# Autodesk Inventor assembly: Сборка апрель
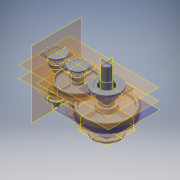
[picture p0: Inventor's stored thumbnail of the model, 180x180]
Saved by Autodesk Inventor 2018 (Build 220112000, 112)
## iProperties
Created: 2018-03-25
Part Number: Сборка апрель
Material: Типовые
Document SubType Name: Assembly
Designer: kriku
Mass: 4694.56 g
Surface Area: 6620.58 cm^2
Volume: 2953.87 cm^3
Density: 1.58929 g/cm^3
Author: kriku
## Documents named in this file (21)
- C:\Users\kriku\OneDrive\Рабочий стол\6 семестр\курсач ДМ\deadmash\Куча инви\Сборка апрель.iam
- C:\Users\kriku\OneDrive\Рабочий стол\6 семестр\курсач ДМ\deadmash\Куча инви\Вал быстроходный.ipt
- C:\Users\kriku\OneDrive\Рабочий стол\6 семестр\курсач ДМ\deadmash\Куча инви\Колесо быстроходное.ipt
- C:\Users\kriku\OneDrive\Рабочий стол\6 семестр\курсач ДМ\deadmash\Куча инви\Вал переходный.ipt
- C:\Users\kriku\OneDrive\Рабочий стол\6 семестр\курсач ДМ\deadmash\Куча инви\Колесл тихоходное.ipt
- C:\Users\kriku\OneDrive\Рабочий стол\6 семестр\курсач ДМ\deadmash\Куча инви\Вал тихоходный.ipt
- C:\Users\kriku\OneDrive\Документы\Inventor\Content Center Files\R2018\ru-RU\GOST 8338-75\Подшипник 206 ГОСТ 8338-75.ipt
- C:\Users\kriku\OneDrive\Документы\Inventor\Content Center Files\R2018\ru-RU\GOST 8338-75\Подшипник 211 ГОСТ 8338-75.ipt
- C:\Users\kriku\OneDrive\Рабочий стол\6 семестр\курсач ДМ\deadmash\Куча инви\Сборка1\Мастер проектирования\Шпоночное соединение1.iam
- C:\Users\kriku\OneDrive\Рабочий стол\6 семестр\курсач ДМ\Куча инви\Крышка обычная на 30.ipt
- C:\Users\kriku\OneDrive\Рабочий стол\6 семестр\курсач ДМ\Куча инви\Крышка обычная на 55.ipt
- C:\Users\kriku\OneDrive\Рабочий стол\6 семестр\курсач ДМ\Куча инви\Крышка сквозная на 55.ipt
- C:\Users\kriku\OneDrive\Документы\Inventor\Content Center Files\R2018\ru-RU\GOST 8752-79(1)\Манжет 1-55x80x8 ГОСТ 8752-79.ipt
- C:\Users\kriku\OneDrive\Рабочий стол\6 семестр\курсач ДМ\Куча инви\Крышка сквозная на 30.ipt
- C:\Users\kriku\OneDrive\Документы\Inventor\Content Center Files\R2018\ru-RU\GOST 8752-79(1)\Манжет 1-30x47x7 ГОСТ 8752-79.ipt
- C:\Users\kriku\OneDrive\Рабочий стол\6 семестр\курсач ДМ\Куча инви\заплечик быстроход больший.ipt
- C:\Users\kriku\OneDrive\Рабочий стол\6 семестр\курсач ДМ\Куча инви\заплечик быстроход меньший.ipt
- C:\Users\kriku\OneDrive\Рабочий стол\6 семестр\курсач ДМ\Куча инви\заплечик переходный.ipt
- C:\Users\kriku\OneDrive\Рабочий стол\6 семестр\курсач ДМ\Куча инви\заплечик переходный  кряком.ipt
- C:\Users\kriku\OneDrive\Рабочий стол\6 семестр\курсач ДМ\Куча инви\заплечикбыстроходный  кряком.ipt
- C:\Users\kriku\OneDrive\Рабочий стол\6 семестр\курсач ДМ\Куча инви\плюс к быстроходному.ipt
## Components (26 placed, 20 different names)
1. Вал быстроходный:1 — Совмещение:1, Совмещение:2, Совмещение:11, Совмещение:12, Совмещение:17, Совмещение:20, Заподлицо:7, Заподлицо:8, Заподлицо:10, Совмещение:36, Цилиндрический:1, Жесткий:1
2. Колесо быстроходное:1 — Заподлицо:1, Совмещение:1, Совмещение:2, Совмещение:3, Совмещение:4, Совмещение:5, Угол:2, С поворотом:5
3. Вал переходный:1 — Совмещение:3, Совмещение:4, Совмещение:5, Совмещение:6, Совмещение:7, Совмещение:8, Совмещение:13, Совмещение:14, Совмещение:18, Совмещение:23, Заподлицо:3, Угол:1, Совмещение:24, Угол:2, Заподлицо:4, Заподлицо:5, Совмещение:26, Заподлицо:6, Совмещение:32, Совмещение:33, Вставка:1
4. Колесл тихоходное:1 — Совмещение:6, Совмещение:7, Совмещение:8, Совмещение:9, Заподлицо:2, Совмещение:10, Совмещение:32, Совмещение:33, С поворотом:3
5. Вал тихоходный:1 — Совмещение:9, Заподлицо:2, Совмещение:10, Совмещение:15, Совмещение:16, Совмещение:19, Совмещение:22, Совмещение:29, Совмещение:30, Совмещение:34, Заподлицо:9
6. Подшипник ГОСТ 8338-75 206:1 — Совмещение:11, Совмещение:17, Совмещение:28, Совмещение:38
7. Подшипник ГОСТ 8338-75 206:2 — Совмещение:12, Совмещение:20, Совмещение:37
8. Подшипник ГОСТ 8338-75 206:3 — Совмещение:13, Совмещение:18, Совмещение:25
9. Подшипник ГОСТ 8338-75 206:4 — Совмещение:14, Совмещение:23, Совмещение:27
10. Подшипник ГОСТ 8338-75 211:1 — Совмещение:15, Совмещение:22, Совмещение:31, С поворотом:4
11. Подшипник ГОСТ 8338-75 211:2 — Совмещение:16, Совмещение:19, Совмещение:35
12. Шпоночное соединение:1 [sub-assembly] — Заподлицо:3, Угол:1, Совмещение:24
13. Крышка обычная на 30:1 — Заподлицо:4, Заподлицо:5, Совмещение:25
14. Крышка обычная на 30:2 — Совмещение:26, Заподлицо:6, Совмещение:27
15. Крышка обычная на 30:3 — Заподлицо:7, Заподлицо:8, Совмещение:28
16. Крышка обычная на 55:1 — Совмещение:29, Совмещение:30, Совмещение:31
17. Крышка сквозная на 55:1 — Совмещение:34, Заподлицо:9, С поворотом:1, Совмещение:35
18. Манжет 1 ГОСТ 8752-79 55 x 80 x 8:1 — С поворотом:1
19. Крышка сквозная на 30:1 — С поворотом:2, Заподлицо:10, Совмещение:36, Совмещение:37
20. Манжет 1 ГОСТ 8752-79 30 x 47 x 7:1 — С поворотом:2
21. заплечик быстроход больший:1 — С поворотом:3
22. заплечик быстроход меньший:1 — С поворотом:4
23. заплечик переходный:1 — С поворотом:5
24. заплечик переходный  кряком:1 — Вставка:1
25. заплечикбыстроходный  кряком:1 — Совмещение:38, Цилиндрический:1
26. плюс к быстроходному:1 — Жесткий:1
## Relationships (58: Mate 37, Flush 11, RevoluteJoint 5, Angle 2, Insert 1, CylindricalJoint 1, WeldJoint 1)
- Заподлицо:1 [Flush]: Колесо быстроходное:1
- Совмещение:1 [Mate] (110 mm): Вал быстроходный:1 ↔ Колесо быстроходное:1
- Совмещение:2 [Mate]: Вал быстроходный:1 ↔ Колесо быстроходное:1
- Совмещение:3 [Mate]: Колесо быстроходное:1 ↔ Вал переходный:1
- Совмещение:4 [Mate]: Колесо быстроходное:1 ↔ Вал переходный:1
- Совмещение:5 [Mate]: Колесо быстроходное:1 ↔ Вал переходный:1
- Совмещение:6 [Mate]: Вал переходный:1 ↔ Колесл тихоходное:1
- Совмещение:7 [Mate]: Вал переходный:1 ↔ Колесл тихоходное:1
- Совмещение:8 [Mate] (150 mm): Вал переходный:1 ↔ Колесл тихоходное:1
- Совмещение:9 [Mate]: Колесл тихоходное:1 ↔ Вал тихоходный:1
- Заподлицо:2 [Flush]: Колесл тихоходное:1 ↔ Вал тихоходный:1
- Совмещение:10 [Mate] (11 mm): Колесл тихоходное:1 ↔ Вал тихоходный:1
- Совмещение:11 [Mate]: Вал быстроходный:1 ↔ Подшипник ГОСТ 8338-75 206:1
- Совмещение:12 [Mate]: Вал быстроходный:1 ↔ Подшипник ГОСТ 8338-75 206:2
- Совмещение:13 [Mate]: Вал переходный:1 ↔ Подшипник ГОСТ 8338-75 206:3
- Совмещение:14 [Mate]: Вал переходный:1 ↔ Подшипник ГОСТ 8338-75 206:4
- Совмещение:15 [Mate]: Вал тихоходный:1 ↔ Подшипник ГОСТ 8338-75 211:1
- Совмещение:16 [Mate]: Вал тихоходный:1 ↔ Подшипник ГОСТ 8338-75 211:2
- Совмещение:17 [Mate]: Вал быстроходный:1 ↔ Подшипник ГОСТ 8338-75 206:1
- Совмещение:18 [Mate]: Вал переходный:1 ↔ Подшипник ГОСТ 8338-75 206:3
- Совмещение:19 [Mate]: Вал тихоходный:1 ↔ Подшипник ГОСТ 8338-75 211:2
- Совмещение:20 [Mate]: Вал быстроходный:1 ↔ Подшипник ГОСТ 8338-75 206:2
- Совмещение:22 [Mate]: Вал тихоходный:1 ↔ Подшипник ГОСТ 8338-75 211:1
- Совмещение:23 [Mate]: Вал переходный:1 ↔ Подшипник ГОСТ 8338-75 206:4
- Заподлицо:3 [Flush] (16 mm): Вал переходный:1 ↔ Шпоночное соединение:1
- Угол:1 [Angle] (180 deg): Вал переходный:1 ↔ Шпоночное соединение:1
- Совмещение:24 [Mate]: Вал переходный:1 ↔ Шпоночное соединение:1
- Угол:2 [Angle] (90 deg): Колесо быстроходное:1 ↔ Вал переходный:1
- Заподлицо:4 [Flush]: Вал переходный:1 ↔ Крышка обычная на 30:1
- Заподлицо:5 [Flush]: Вал переходный:1 ↔ Крышка обычная на 30:1
- Совмещение:25 [Mate]: Подшипник ГОСТ 8338-75 206:3 ↔ Крышка обычная на 30:1
- Совмещение:26 [Mate]: Вал переходный:1 ↔ Крышка обычная на 30:2
- Заподлицо:6 [Flush]: Вал переходный:1 ↔ Крышка обычная на 30:2
- Совмещение:27 [Mate]: Подшипник ГОСТ 8338-75 206:4 ↔ Крышка обычная на 30:2
- Заподлицо:7 [Flush]: Вал быстроходный:1 ↔ Крышка обычная на 30:3
- Заподлицо:8 [Flush]: Вал быстроходный:1 ↔ Крышка обычная на 30:3
- Совмещение:28 [Mate]: Подшипник ГОСТ 8338-75 206:1 ↔ Крышка обычная на 30:3
- Совмещение:29 [Mate]: Вал тихоходный:1 ↔ Крышка обычная на 55:1
- Совмещение:30 [Mate]: Вал тихоходный:1 ↔ Крышка обычная на 55:1
- Совмещение:31 [Mate]: Подшипник ГОСТ 8338-75 211:1 ↔ Крышка обычная на 55:1
- Совмещение:32 [Mate]: Вал переходный:1 ↔ Колесл тихоходное:1
- Совмещение:33 [Mate]: Вал переходный:1 ↔ Колесл тихоходное:1
- Совмещение:34 [Mate]: Вал тихоходный:1 ↔ Крышка сквозная на 55:1
- Заподлицо:9 [Flush]: Вал тихоходный:1 ↔ Крышка сквозная на 55:1
- С поворотом:1 [RevoluteJoint]: Крышка сквозная на 55:1 ↔ Манжет 1 ГОСТ 8752-79 55 x 80 x 8:1
- Совмещение:35 [Mate]: Подшипник ГОСТ 8338-75 211:2 ↔ Крышка сквозная на 55:1
- С поворотом:2 [RevoluteJoint]: Крышка сквозная на 30:1 ↔ Манжет 1 ГОСТ 8752-79 30 x 47 x 7:1
- Заподлицо:10 [Flush]: Вал быстроходный:1 ↔ Крышка сквозная на 30:1
- Совмещение:36 [Mate]: Вал быстроходный:1 ↔ Крышка сквозная на 30:1
- Совмещение:37 [Mate]: Подшипник ГОСТ 8338-75 206:2 ↔ Крышка сквозная на 30:1
- С поворотом:3 [RevoluteJoint]: Колесл тихоходное:1 ↔ заплечик быстроход больший:1
- С поворотом:4 [RevoluteJoint]: Подшипник ГОСТ 8338-75 211:1 ↔ заплечик быстроход меньший:1
- С поворотом:5 [RevoluteJoint]: Колесо быстроходное:1 ↔ заплечик переходный:1
- Вставка:1 [Insert]: Вал переходный:1 ↔ заплечик переходный  кряком:1
- Совмещение:38 [Mate]: Подшипник ГОСТ 8338-75 206:1 ↔ заплечикбыстроходный  кряком:1
- Цилиндрический:1 [CylindricalJoint]: Вал быстроходный:1 ↔ заплечикбыстроходный  кряком:1
- Жесткий:1 [WeldJoint]: Вал быстроходный:1 ↔ плюс к быстроходному:1
- Заподлицо:11 [Flush] (60 mm)
